# Autodesk Inventor assembly: innerhub_assembly
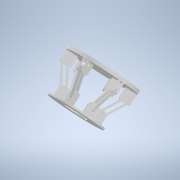
[picture p0: Inventor's stored thumbnail of the model, 180x180]
Saved by Autodesk Inventor 2020 (Build 240168000, 168)
## iProperties
Created: 2019-09-23
Part Number: innerhub_assembly
Document SubType Name: Assembly
Designer: dlr6513
Author: dlr6513
## Documents named in this file (5)
- C:\Users\dlr6513\Desktop\ADABot_CAD\innerhub_assembly.iam
- C:\Users\dlr6513\Desktop\ADABot_CAD\inner_hub.ipt
- C:\Users\dlr6513\Desktop\ADABot_CAD\extention_rod.ipt
- C:\Users\dlr6513\Desktop\ADABot_CAD\extention_plate.ipt
- C:\Users\dlr6513\Desktop\ADABot_CAD\outer_hub.ipt
## Components (20 placed, 4 different names)
1. inner_hub:1 — Mate:1, Flush:1, Flush:2, Mate:4, Flush:3, Mate:6, Mate:7, Mate:9, Flush:4, Mate:12, Mate:13, Flush:6, Mate:15, Mate:16, Flush:7, Mate:17, Flush:8, Mate:19, Mate:21, Mate:24
2. extention_rod:1 — Mate:1, Flush:1, Flush:2, Mate:5
3. extention_rod:2 — Mate:4, Flush:3, Mate:8
4. extention_plate:1 — Mate:5, Mate:6, Tangent:4
5. extention_plate:2 — Mate:7, Mate:8, Tangent:7
6. extention_plate:3 — Mate:18, Mate:19, Tangent:3
7. extention_plate:4 — Mate:11, Mate:12, Tangent:5
8. extention_plate:6 — Mate:14, Mate:15, Tangent:6
9. extention_rod:3 — Mate:13, Flush:6, Mate:14
10. extention_rod:4 — Mate:9, Flush:4, Mate:11
11. extention_rod:5 — Mate:16, Flush:7, Mate:20
12. extention_rod:6 — Mate:10, Flush:5
13. outer_hub:1 — Mate:10, Flush:5, Mate:23, Tangent:2, Mate:24, Tangent:3, Tangent:4, Tangent:5, Tangent:6, Tangent:7, Flush:9, Mate:25, Flush:10, Mate:26, Mate:27, Flush:11, Mate:28, Flush:12, Mate:29, Flush:13
14. extention_rod:7 — Mate:17, Flush:8, Mate:18
15. extention_plate:7 — Mate:20, Mate:21, Mate:23, Tangent:2
16. extention_rod:8 — Mate:28, Flush:12
17. extention_rod:9 — Flush:9, Mate:25
18. extention_rod:10 — Mate:27, Flush:11
19. extention_rod:11 — Flush:10, Mate:26
20. extention_rod:12 — Mate:29, Flush:13
## Relationships (45: Mate 26, Flush 13, Tangent 6)
- Mate:1: inner_hub:1 ↔ extention_rod:1
- Flush:1: inner_hub:1 ↔ extention_rod:1
- Flush:2: inner_hub:1 ↔ extention_rod:1
- Mate:4: inner_hub:1 ↔ extention_rod:2
- Flush:3: inner_hub:1 ↔ extention_rod:2
- Mate:5: extention_rod:1 ↔ extention_plate:1
- Mate:6: inner_hub:1 ↔ extention_plate:1
- Mate:7: inner_hub:1 ↔ extention_plate:2
- Mate:8: extention_rod:2 ↔ extention_plate:2
- Mate:9: inner_hub:1 ↔ extention_rod:4
- Flush:4: inner_hub:1 ↔ extention_rod:4
- Mate:10: extention_rod:6 ↔ outer_hub:1
- Flush:5: extention_rod:6 ↔ outer_hub:1
- Mate:11: extention_plate:4 ↔ extention_rod:4
- Mate:12: inner_hub:1 ↔ extention_plate:4
- Mate:13: inner_hub:1 ↔ extention_rod:3
- Flush:6: inner_hub:1 ↔ extention_rod:3
- Mate:14: extention_plate:6 ↔ extention_rod:3
- Mate:15: inner_hub:1 ↔ extention_plate:6
- Mate:16: inner_hub:1 ↔ extention_rod:5
- Flush:7: inner_hub:1 ↔ extention_rod:5
- Mate:17: inner_hub:1 ↔ extention_rod:7
- Flush:8: inner_hub:1 ↔ extention_rod:7
- Mate:18: extention_plate:3 ↔ extention_rod:7
- Mate:19: inner_hub:1 ↔ extention_plate:3
- Mate:20: extention_rod:5 ↔ extention_plate:7
- Mate:21: inner_hub:1 ↔ extention_plate:7
- Mate:23: outer_hub:1 ↔ extention_plate:7
- Tangent:2: outer_hub:1 ↔ extention_plate:7
- Mate:24: inner_hub:1 ↔ outer_hub:1
- Tangent:3: extention_plate:3 ↔ outer_hub:1
- Tangent:4: extention_plate:1 ↔ outer_hub:1
- Tangent:5: extention_plate:4 ↔ outer_hub:1
- Tangent:6: extention_plate:6 ↔ outer_hub:1
- Tangent:7: extention_plate:2 ↔ outer_hub:1
- Flush:9: outer_hub:1 ↔ extention_rod:9
- Mate:25: outer_hub:1 ↔ extention_rod:9
- Flush:10: outer_hub:1 ↔ extention_rod:11
- Mate:26: outer_hub:1 ↔ extention_rod:11
- Mate:27: outer_hub:1 ↔ extention_rod:10
- Flush:11: outer_hub:1 ↔ extention_rod:10
- Mate:28: outer_hub:1 ↔ extention_rod:8
- Flush:12: outer_hub:1 ↔ extention_rod:8
- Mate:29: outer_hub:1 ↔ extention_rod:12
- Flush:13: outer_hub:1 ↔ extention_rod:12
